# Autodesk Inventor assembly: Hand Assembly
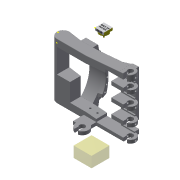
[picture p0: Inventor's stored thumbnail of the model, 180x180]
Saved by Autodesk Inventor 2017 (Build 210142000, 142)
## iProperties
Created: 2016-09-28
Part Number: Hand Assembly
Document SubType Name: Assembly
Designer: cmcdona
Author: cmcdona
## Documents named in this file (9)
- D:\cmcdona\My Research\Documents\Open\McMaster\Engineering 1\Courses\2016-17\T1 - ENG 1C03\Project\Project Files\Hand Assembly.iam
- D:\cmcdona\My Research\Documents\Open\McMaster\Engineering 1\Courses\2016-17\T1 - ENG 1C03\Project\Project Files\Hand - Frame.ipt
- D:\cmcdona\My Research\Documents\Open\McMaster\Engineering 1\Courses\2016-17\T1 - ENG 1C03\Project\Project Files\Hand - Digit 4.ipt
- D:\cmcdona\My Research\Documents\Open\McMaster\Engineering 1\Courses\2016-17\T1 - ENG 1C03\Project\Project Files\Hand - Digit 0-1.ipt
- D:\cmcdona\My Research\Documents\Open\McMaster\Engineering 1\Courses\2016-17\T1 - ENG 1C03\Project\Project Files\Hand - Distal Bridge.ipt
- D:\cmcdona\My Research\Documents\Open\McMaster\Engineering 1\Courses\2016-17\T1 - ENG 1C03\Project\Project Files\Hand - Digit 2-3.ipt
- D:\cmcdona\My Research\Documents\Open\McMaster\Engineering 1\Courses\2016-17\T1 - ENG 1C03\Project\Project Files\Hand - Proximal Bridge.ipt
- D:\cmcdona\My Research\Documents\Open\McMaster\Engineering 1\Courses\2016-17\T1 - ENG 1C03\Project\Project Files\Hand - Functional Workspace.ipt
- D:\cmcdona\My Research\Documents\Open\McMaster\Engineering 1\Courses\2016-17\T1 - ENG 1C03\Project\Project Files\Input Motor.ipt
## Components (10 placed, 8 different names)
1. Hand - Frame:1 — Flush:1, Flush:2, Mate:1, Mate:2, Flush:3, Mate:3, Mate:16, Mate:17, Mate:18
2. Hand - Digit 4:1 — Flush:1, Flush:2, Mate:1, Mate:4, Mate:5
3. Hand - Digit 0-1:1 — Mate:2, Flush:3, Mate:3, Mate:6, Mate:19, Mate:20, Mate:21
4. Hand - Distal Bridge:1 — Mate:4, Mate:5, Mate:6, Mate:7, Mate:8, Mate:9, Mate:10, Mate:11, Mate:12, Mate:13, Mate:14, Mate:15
5. Hand - Digit 2-3:1 — Mate:7, Mate:8, Mate:9
6. Hand - Digit 2-3:2 — Mate:10, Mate:11, Mate:12
7. Hand - Digit 2-3:3 — Mate:13, Mate:14, Mate:15
8. Hand - Proximal Bridge:1 — Mate:16, Mate:17, Mate:18
9. Hand - Functional Workspace:1 — Mate:19, Mate:20, Mate:21
10. Input Motor:1
## Relationships (24: Mate 21, Flush 3)
- Flush:1: Hand - Frame:1 ↔ Hand - Digit 4:1
- Flush:2: Hand - Frame:1 ↔ Hand - Digit 4:1
- Mate:1: Hand - Frame:1 ↔ Hand - Digit 4:1
- Mate:2: Hand - Frame:1 ↔ Hand - Digit 0-1:1
- Flush:3: Hand - Frame:1 ↔ Hand - Digit 0-1:1
- Mate:3: Hand - Frame:1 ↔ Hand - Digit 0-1:1
- Mate:4: Hand - Digit 4:1 ↔ Hand - Distal Bridge:1
- Mate:5: Hand - Digit 4:1 ↔ Hand - Distal Bridge:1
- Mate:6: Hand - Digit 0-1:1 ↔ Hand - Distal Bridge:1
- Mate:7: Hand - Distal Bridge:1 ↔ Hand - Digit 2-3:1
- Mate:8: Hand - Distal Bridge:1 ↔ Hand - Digit 2-3:1
- Mate:9: Hand - Distal Bridge:1 ↔ Hand - Digit 2-3:1
- Mate:10: Hand - Distal Bridge:1 ↔ Hand - Digit 2-3:2
- Mate:11: Hand - Distal Bridge:1 ↔ Hand - Digit 2-3:2
- Mate:12: Hand - Distal Bridge:1 ↔ Hand - Digit 2-3:2
- Mate:13: Hand - Distal Bridge:1 ↔ Hand - Digit 2-3:3
- Mate:14: Hand - Distal Bridge:1 ↔ Hand - Digit 2-3:3
- Mate:15: Hand - Distal Bridge:1 ↔ Hand - Digit 2-3:3
- Mate:16: Hand - Frame:1 ↔ Hand - Proximal Bridge:1
- Mate:17: Hand - Frame:1 ↔ Hand - Proximal Bridge:1
- Mate:18: Hand - Frame:1 ↔ Hand - Proximal Bridge:1
- Mate:19: Hand - Digit 0-1:1 ↔ Hand - Functional Workspace:1
- Mate:20 (41 mm): Hand - Digit 0-1:1 ↔ Hand - Functional Workspace:1
- Mate:21 (33 mm): Hand - Digit 0-1:1 ↔ Hand - Functional Workspace:1
